# Autodesk Inventor assembly: Allen&Cap
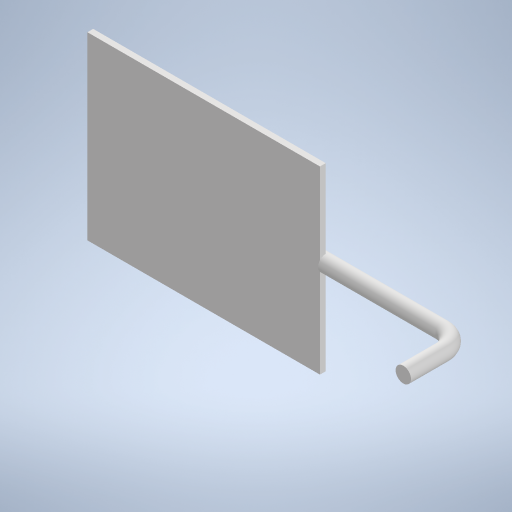
[picture p0: Inventor's stored thumbnail of the model, 512x512]
Saved by Autodesk Inventor 2024.3 (Build 283343000, 343)
## iProperties
Created: 2025-08-10
Part Number: Allen&Cap
Document SubType Name: Assembly
Designer: ajclo
Author: ajclo
## Documents named in this file (3)
- C:\Users\ajclo\OneDrive - Stellenbosch University\Documents\BEng\Year IV\Skripsie\CAD\CAD Final Design\Allen&Cap.iam
- C:\Users\ajclo\OneDrive - Stellenbosch University\Documents\BEng\Year IV\Skripsie\CAD\CAD Final Design\AllenKey-RS3.ipt
- C:\Users\ajclo\OneDrive - Stellenbosch University\Documents\BEng\Year IV\Skripsie\CAD\CAD Final Design\CapRS3.ipt
## Components (2 placed, 2 different names)
1. AllenKey-RS3:1 — Mate:1, Mate:2, Mate:3
2. CapRS3:1 — Mate:1, Mate:2, Mate:3
## Relationships (3: Mate 3)
- Mate:1: AllenKey-RS3:1 ↔ CapRS3:1
- Mate:2: AllenKey-RS3:1 ↔ CapRS3:1
- Mate:3 (44.5 mm): AllenKey-RS3:1 ↔ CapRS3:1
